# Autodesk Inventor assembly: Electronics Chassis
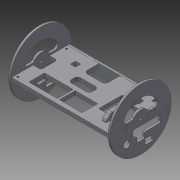
[picture p0: Inventor's stored thumbnail of the model, 180x180]
Saved by Autodesk Inventor 2015 (Build 190159000, 159)
## iProperties
Created: 2015-06-17
Part Number: Electronics Chassis
Document SubType Name: Assembly
Designer: JR
Author: JR
## Documents named in this file (5)
- F:\OpenROV\2.8\Electronics Tube\Aft\Electronics Chassis.iam
- F:\OpenROV\2.8\Electronics Tube\Aft\Electronics Chassis Main 6mm.ipt
- F:\OpenROV\2.8\Electronics Tube\Aft\Electronics Chassis Servo Mount.ipt
- F:\OpenROV\2.8\Electronics Tube\Aft\Electronics Chassis Side.ipt
- F:\OpenROV\2.8\Electronics Tube\Aft\Electronics Chassis Wall.ipt
## Components (5 placed, 4 different names)
1. Electronics Chassis Main 6mm:1 — Mate:1, Mate:2, Flush:1, Mate:6, Mate:7, Mate:8, Mate:9, Mate:10, Mate:11, Mate:12, Mate:13, Mate:14
2. Electronics Chassis Servo Mount:1 — Mate:12, Mate:13, Mate:14
3. Electronics Chassis Side:1 — Mate:6, Mate:7, Mate:8
4. Electronics Chassis Side:2 — Mate:9, Mate:10, Mate:11
5. Electronics Chassis Wall:1 — Mate:1, Mate:2, Flush:1
## Relationships (12: Mate 11, Flush 1)
- Mate:1: Electronics Chassis Main 6mm:1 ↔ Electronics Chassis Wall:1
- Mate:2: Electronics Chassis Main 6mm:1 ↔ Electronics Chassis Wall:1
- Flush:1: Electronics Chassis Main 6mm:1 ↔ Electronics Chassis Wall:1
- Mate:6: Electronics Chassis Main 6mm:1 ↔ Electronics Chassis Side:1
- Mate:7: Electronics Chassis Main 6mm:1 ↔ Electronics Chassis Side:1
- Mate:8: Electronics Chassis Main 6mm:1 ↔ Electronics Chassis Side:1
- Mate:9: Electronics Chassis Main 6mm:1 ↔ Electronics Chassis Side:2
- Mate:10: Electronics Chassis Main 6mm:1 ↔ Electronics Chassis Side:2
- Mate:11: Electronics Chassis Main 6mm:1 ↔ Electronics Chassis Side:2
- Mate:12: Electronics Chassis Main 6mm:1 ↔ Electronics Chassis Servo Mount:1
- Mate:13: Electronics Chassis Main 6mm:1 ↔ Electronics Chassis Servo Mount:1
- Mate:14: Electronics Chassis Main 6mm:1 ↔ Electronics Chassis Servo Mount:1
